# Autodesk Inventor assembly: frontAssembly
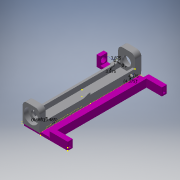
[picture p0: Inventor's stored thumbnail of the model, 180x180]
Saved by Autodesk Inventor 2018 (Build 220112000, 112)
## iProperties
Created: 2019-04-30
Part Number: frontAssembly
Document SubType Name: Assembly
Designer: Aditya Kendre
Author: Aditya Kendre
## Documents named in this file (3)
- C:\Users\Aditya Kendre\Documents\JibCar\frontAssembly.iam
- C:\Users\Aditya Kendre\Documents\JibCar\mtv_frontAxelHolder(4_30).ipt
- C:\Users\Aditya Kendre\Documents\JibCar\mtv_frontHolder(4_30).ipt
## Components (2 placed, 2 different names)
1. mtv_frontAxelHolder(4_30):1 — Mate:1
2. mtv_frontHolder(4_30):1 — Mate:1
## Relationships (1: Mate 1)
- Mate:1: mtv_frontAxelHolder(4_30):1 ↔ mtv_frontHolder(4_30):1
